# Autodesk Inventor assembly: gear_7
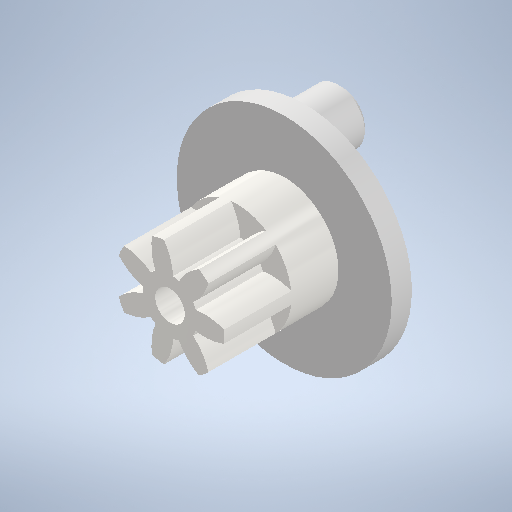
[picture p0: Inventor's stored thumbnail of the model, 512x512]
Saved by Autodesk Inventor 2025 (Build 290162000, 162)
## iProperties
Created: 2025-10-23
Part Number: gear_7
Document SubType Name: Assembly
Designer: sooo1
Author: sooo1
## Documents named in this file (3)
- C:\Users\sooo1\Documents\Inventor\MOBITOUCH\final\stroke_module_1\gear_7.iam
- C:\Users\sooo1\Documents\Inventor\MOBITOUCH\final\stroke_module_1\adapter_xl320.ipt
- C:\Users\sooo1\Documents\Inventor\MOBITOUCH\final\stroke_module_1\gear_7\デザイン アクセラレータ\平歯車12.ipt
## Components (2 placed, 2 different names)
1. adapter_xl320:1 — フラッシュ:1, フラッシュ:2, フラッシュ:3, フラッシュ:4, メイト:3, メイト:4
2. 平歯車1:1 — メイト:3, メイト:4, メイト:5
## Relationships (7: Flush 4, Mate 3)
- フラッシュ:1 [Flush]: adapter_xl320:1
- フラッシュ:2 [Flush]: adapter_xl320:1
- フラッシュ:3 [Flush]: adapter_xl320:1
- フラッシュ:4 [Flush]: adapter_xl320:1
- メイト:3 [Mate]: adapter_xl320:1 ↔ 平歯車1:1
- メイト:4 [Mate]: adapter_xl320:1 ↔ 平歯車1:1
- メイト:5 [Mate]: 平歯車1:1
